# Autodesk Inventor assembly: USB_Assem
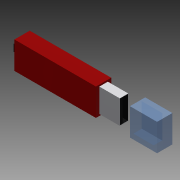
[picture p0: Inventor's stored thumbnail of the model, 180x180]
Saved by Autodesk Inventor 2015 (Build 190159000, 159)
## iProperties
Created: 2015-02-01
Part Number: USB_Assem
Document SubType Name: Assembly
Designer: Paul
Author: Paul
## Documents named in this file (3)
- C:\Users\paul\Google Drive\All #ResBaz Shared\Paul2AlizaCAD\06_Assembly\01_USB_Assembly\USB_Assem_Answer.iam
- C:\Users\paul\Google Drive\All #ResBaz Shared\Paul2AlizaCAD\06_Assembly\01_USB_Assembly\USB_Stick.ipt
- C:\Users\paul\Google Drive\All #ResBaz Shared\Paul2AlizaCAD\06_Assembly\01_USB_Assembly\USB_Cap.ipt
## Components (2 placed, 2 different names)
1. USB_Stick:1 — Flush:1, Flush:2, Mate:1
2. USB_Cap:1 — Flush:1, Flush:2, Mate:1
## Relationships (3: Flush 2, Mate 1)
- Flush:1: USB_Stick:1 ↔ USB_Cap:1
- Flush:2: USB_Stick:1 ↔ USB_Cap:1
- Mate:1 (20 mm): USB_Stick:1 ↔ USB_Cap:1
